# Autodesk Inventor assembly: wildfire
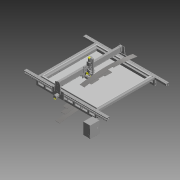
[picture p0: Inventor's stored thumbnail of the model, 180x180]
Saved by Autodesk Inventor 2013 (Build 170138000, 138)
## iProperties
Created: 2012-11-30
Part Number: wildfire
Document SubType Name: Assembly
Designer: istvan.burbank
Mass: 35060.2 g
Surface Area: 149069 cm^2
Volume: 21794.8 cm^3
Density: 1.60865 g/cm^3
Author: istvan.burbank
## Documents named in this file (10)
- C:\Users\istvan.burbank\Documents\GitHub\Crown-Fire\CAD\wildfire.iam
- C:\Users\istvan.burbank\Documents\GitHub\Crown-Fire\CAD\Frame\frame.iam
- C:\Users\istvan.burbank\Documents\GitHub\Crown-Fire\CAD\GantryMount\tractor.iam
- C:\Users\istvan.burbank\Documents\GitHub\Crown-Fire\CAD\Gantry\gantry.iam
- C:\Users\istvan.burbank\Documents\GitHub\Crown-Fire\CAD\Carriage\carriage.iam
- C:\Users\istvan.burbank\Documents\GitHub\Crown-Fire\CAD\CuttingHead\CuttingHead.iam
- C:\Users\istvan.burbank\Documents\GitHub\Crown-Fire\CAD\Torch\machineTorchHead.ipt
- C:\Users\istvan.burbank\Documents\GitHub\Crown-Fire\CAD\Electronics\wildfire.Harness.iam
- C:\Users\istvan.burbank\Documents\GitHub\Crown-Fire\CAD\Electronics\ControlBox.iam
- C:\Users\istvan.burbank\Documents\GitHub\Crown-Fire\CAD\Electronics\Connectors\db9-male.ipt
## Components (13 placed, 9 different names)
1. frame:1 [sub-assembly] — Tangent:13, Tangent:14, Tangent:15, Tangent:16, Tangent:17
2. tractor:1 [sub-assembly] — Mate:8, Mate:9, Tangent:16, Tangent:17
3. tractor:2 [sub-assembly] — Mate:4, Mate:6, Mate:7, Tangent:13, Tangent:14, Tangent:15
4. gantry:1 [sub-assembly] — Mate:4, Mate:6, Mate:7, Mate:8, Mate:9, Tangent:10, Tangent:11, Tangent:12
5. carriage:1 [sub-assembly] — Mate:10, Angle:1, Tangent:10, Tangent:11, Tangent:12
6. CuttingHead:1 [sub-assembly] — Mate:10, Angle:1, Mate:13, Flush:1
7. machineTorchHead:1 — Mate:13, Flush:1
8. wildfire.Harness [sub-assembly]
9. ControlBox:1 [sub-assembly] — Mate:14, Mate:15, Angle:2, Mate:16, Mate:17, Mate:18, Mate:20, Mate:21, Mate:22, Angle:3, Angle:4, Angle:5
10. db9-male:1 — Mate:14, Mate:15, Angle:2
11. db9-male:2 — Mate:18, Mate:21, Angle:5
12. db9-male:3 — Mate:17, Mate:20, Angle:4
13. db9-male:4 — Mate:16, Mate:22, Angle:3
## Relationships (29: Mate 15, Tangent 8, Angle 5, Flush 1)
- Mate:4: tractor:2 ↔ gantry:1
- Mate:6: tractor:2 ↔ gantry:1
- Mate:7: tractor:2 ↔ gantry:1
- Mate:8: tractor:1 ↔ gantry:1
- Mate:9: tractor:1 ↔ gantry:1
- Mate:10: carriage:1 ↔ CuttingHead:1
- Angle:1 (0 deg): carriage:1 ↔ CuttingHead:1
- Mate:13: CuttingHead:1 ↔ machineTorchHead:1
- Flush:1 (-57.15 mm): CuttingHead:1 ↔ machineTorchHead:1
- Tangent:10: gantry:1 ↔ carriage:1
- Tangent:11: gantry:1 ↔ carriage:1
- Tangent:12: gantry:1 ↔ carriage:1
- Tangent:13: frame:1 ↔ tractor:2
- Tangent:14: frame:1 ↔ tractor:2
- Tangent:15: frame:1 ↔ tractor:2
- Tangent:16: frame:1 ↔ tractor:1
- Tangent:17: frame:1 ↔ tractor:1
- Mate:14: ControlBox:1 ↔ db9-male:1
- Mate:15: ControlBox:1 ↔ db9-male:1
- Angle:2 (0 deg): ControlBox:1 ↔ db9-male:1
- Mate:16: ControlBox:1 ↔ db9-male:4
- Mate:17: ControlBox:1 ↔ db9-male:3
- Mate:18: ControlBox:1 ↔ db9-male:2
- Mate:20: ControlBox:1 ↔ db9-male:3
- Mate:21: ControlBox:1 ↔ db9-male:2
- Mate:22: ControlBox:1 ↔ db9-male:4
- Angle:3 (0 deg): ControlBox:1 ↔ db9-male:4
- Angle:4 (0 deg): ControlBox:1 ↔ db9-male:3
- Angle:5 (0 deg): ControlBox:1 ↔ db9-male:2
